# Autodesk Inventor assembly: deskShelf
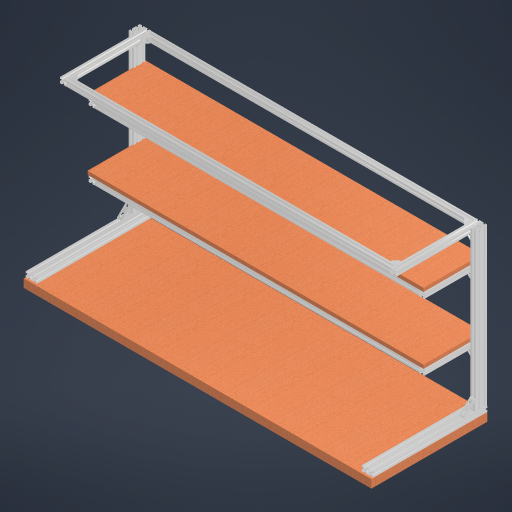
[picture p0: Inventor's stored thumbnail of the model, 512x512]
Saved by Autodesk Inventor 2023 (Build 270158000, 158)
## iProperties
Created: 2023-03-26
Part Number: deskShelf
Document SubType Name: Assembly
Designer: austi
Author: austi
## Documents named in this file (11)
- E:\OneDrive\work\deepSpaceEngineering\deskShelf.iam
- E:\OneDrive\work\deepSpaceEngineering\Part1.ipt
- E:\OneDrive\work\deepSpaceEngineering\shelf.ipt
- E:\OneDrive\work\deepSpaceEngineering\30-3030-1708-CL.ipt
- E:\OneDrive\work\deepSpaceEngineering\30-3060-825-CL.ipt
- E:\OneDrive\work\deepSpaceEngineering\30-3060-600-CL.ipt
- E:\OneDrive\work\deepSpaceEngineering\30-3030-300-CL.ipt
- E:\OneDrive\work\deepSpaceEngineering\30-3030-450-CL.ipt
- E:\OneDrive\work\deepSpaceEngineering\30-4336_Aluminum.ipt
- E:\OneDrive\work\deepSpaceEngineering\30-4134_Aluminum.ipt
- E:\OneDrive\work\deepSpaceEngineering\14073.ipt
## Components (39 placed, 10 different names)
1. Part1:1 — Mate:1, Flush:2, Flush:3, Mate:2, Mate:6, Mate:8, Flush:32
2. shelf:1 — Mate:63, Flush:51, Flush:52
3. shelf:2 — Mate:62, Flush:49, Flush:50
4. 30-3030-1708-CL:1 — Mate:11, Flush:12, Flush:13, Mate:49, Flush:42, Mate:56, Flush:46, Flush:49
5. 30-3030-1708-CL:2 — Flush:10, Mate:9, Flush:11, Mate:10, Flush:37, Mate:39, Mate:51, Mate:62
6. 30-3030-1708-CL:4 — Mate:17, Flush:18, Flush:19, Mate:47, Flush:41, Mate:58, Flush:47, Mate:63, Flush:52
7. 30-3030-1708-CL:6 — Mate:16, Flush:16, Flush:17, Mate:41, Mate:53
8. 30-3060-825-CL:1 — Mate:3, Flush:4, Flush:5, Mate:5, Flush:8, Mate:12, Flush:14, Mate:18, Flush:20, Flush:21, Mate:23, Flush:28, Mate:26, Mate:28, Flush:31, Mate:30
9. 30-3060-825-CL:2 — Mate:4, Flush:6, Flush:7, Flush:9, Mate:7, Mate:14, Flush:15, Mate:19, Flush:22, Flush:23, Mate:25, Flush:29, Mate:32, Flush:34, Mate:34, Flush:35, Mate:36, Flush:36
10. 30-3060-600-CL:1 — Mate:1, Flush:2, Mate:3, Flush:4, Flush:5, Mate:22, Flush:32
11. 30-3060-600-CL:2 — Flush:3, Mate:2, Mate:4, Flush:6, Flush:7, Mate:24
12. 30-3030-300-CL:1 — Mate:5, Flush:8, Mate:6, Mate:10, Mate:11, Flush:12, Flush:13, Mate:13, Mate:27, Flush:30, Mate:38, Mate:48, Flush:50
13. 30-3030-300-CL:2 — Mate:14, Flush:15, Mate:15, Mate:16, Flush:16, Flush:17, Mate:17, Flush:18, Flush:19, Mate:35, Mate:52, Flush:44, Mate:59
14. 30-3030-300-CL:3 — Mate:12, Flush:14, Mate:13, Mate:29, Mate:40, Flush:38, Mate:46, Flush:51
15. 30-3030-300-CL:4 — Flush:9, Mate:7, Mate:8, Flush:10, Mate:9, Flush:11, Mate:15, Mate:33, Mate:50, Flush:43, Mate:57
16. 30-3030-450-CL:1 — Mate:18, Flush:20, Flush:21, Mate:20, Flush:24, Flush:25, Mate:21, Flush:26, Flush:27, Mate:31, Flush:33, Mate:42, Flush:39, Mate:44
17. 30-3030-450-CL:2 — Mate:19, Flush:22, Flush:23, Mate:37, Mate:54, Flush:45, Mate:61
18. 30-3030-1708-CL:7 — Mate:21, Flush:26, Flush:27, Mate:43, Mate:55
19. 30-3030-1708-CL:8 — Mate:20, Flush:24, Flush:25, Mate:45, Flush:40, Mate:60, Flush:48
20. 30-4336_Aluminum:1 — Mate:22, Mate:23, Flush:28
21. 30-4336_Aluminum:2 — Mate:24, Mate:25, Flush:29
22. 30-4134_Aluminum:1 — Mate:32, Mate:33, Flush:34
23. 30-4134_Aluminum:2 — Mate:34, Mate:35, Flush:35
24. 30-4134_Aluminum:3 — Mate:36, Mate:37, Flush:36
25. 30-4134_Aluminum:4 — Mate:30, Mate:31, Flush:33
26. 30-4134_Aluminum:5 — Mate:28, Flush:31, Mate:29
27. 30-4134_Aluminum:6 — Mate:26, Mate:27, Flush:30
28. 14073:1 — Mate:38, Flush:37, Mate:39
29. 14073:2 — Mate:40, Flush:38, Mate:41
30. 14073:3 — Mate:42, Flush:39, Mate:43
31. 14073:4 — Mate:50, Mate:51, Flush:43
32. 14073:5 — Mate:52, Mate:53, Flush:44
33. 14073:6 — Mate:54, Mate:55, Flush:45
34. 14073:7 — Mate:56, Mate:57, Flush:46
35. 14073:8 — Mate:58, Mate:59, Flush:47
36. 14073:9 — Mate:60, Mate:61, Flush:48
37. 14073:10 — Mate:44, Mate:45, Flush:40
38. 14073:11 — Mate:48, Mate:49, Flush:42
39. 14073:12 — Mate:46, Mate:47, Flush:41
## Relationships (114: Mate 63, Flush 51)
- Mate:1: Part1:1 ↔ 30-3060-600-CL:1
- Flush:2: Part1:1 ↔ 30-3060-600-CL:1
- Flush:3: Part1:1 ↔ 30-3060-600-CL:2
- Mate:2: Part1:1 ↔ 30-3060-600-CL:2
- Mate:3: 30-3060-825-CL:1 ↔ 30-3060-600-CL:1
- Flush:4: 30-3060-825-CL:1 ↔ 30-3060-600-CL:1
- Flush:5: 30-3060-825-CL:1 ↔ 30-3060-600-CL:1
- Mate:4: 30-3060-825-CL:2 ↔ 30-3060-600-CL:2
- Flush:6: 30-3060-825-CL:2 ↔ 30-3060-600-CL:2
- Flush:7: 30-3060-825-CL:2 ↔ 30-3060-600-CL:2
- Mate:5: 30-3060-825-CL:1 ↔ 30-3030-300-CL:1
- Flush:8: 30-3060-825-CL:1 ↔ 30-3030-300-CL:1
- Mate:6 (300 mm): Part1:1 ↔ 30-3030-300-CL:1
- Flush:9: 30-3060-825-CL:2 ↔ 30-3030-300-CL:4
- Mate:7: 30-3060-825-CL:2 ↔ 30-3030-300-CL:4
- Mate:8 (300 mm): Part1:1 ↔ 30-3030-300-CL:4
- Flush:10: 30-3030-1708-CL:2 ↔ 30-3030-300-CL:4
- Mate:9: 30-3030-1708-CL:2 ↔ 30-3030-300-CL:4
- Flush:11: 30-3030-1708-CL:2 ↔ 30-3030-300-CL:4
- Mate:10: 30-3030-1708-CL:2 ↔ 30-3030-300-CL:1
- Mate:11: 30-3030-1708-CL:1 ↔ 30-3030-300-CL:1
- Flush:12: 30-3030-1708-CL:1 ↔ 30-3030-300-CL:1
- Flush:13: 30-3030-1708-CL:1 ↔ 30-3030-300-CL:1
- Mate:12: 30-3060-825-CL:1 ↔ 30-3030-300-CL:3
- Flush:14: 30-3060-825-CL:1 ↔ 30-3030-300-CL:3
- Mate:13 (320 mm): 30-3030-300-CL:1 ↔ 30-3030-300-CL:3
- Mate:14: 30-3060-825-CL:2 ↔ 30-3030-300-CL:2
- Flush:15: 30-3060-825-CL:2 ↔ 30-3030-300-CL:2
- Mate:15 (320 mm): 30-3030-300-CL:2 ↔ 30-3030-300-CL:4
- Mate:16: 30-3030-1708-CL:6 ↔ 30-3030-300-CL:2
- Flush:16: 30-3030-1708-CL:6 ↔ 30-3030-300-CL:2
- Flush:17: 30-3030-1708-CL:6 ↔ 30-3030-300-CL:2
- Mate:17: 30-3030-1708-CL:4 ↔ 30-3030-300-CL:2
- Flush:18: 30-3030-1708-CL:4 ↔ 30-3030-300-CL:2
- Flush:19: 30-3030-1708-CL:4 ↔ 30-3030-300-CL:2
- Mate:18: 30-3060-825-CL:1 ↔ 30-3030-450-CL:1
- Flush:20: 30-3060-825-CL:1 ↔ 30-3030-450-CL:1
- Flush:21: 30-3060-825-CL:1 ↔ 30-3030-450-CL:1
- Mate:19: 30-3060-825-CL:2 ↔ 30-3030-450-CL:2
- Flush:22: 30-3060-825-CL:2 ↔ 30-3030-450-CL:2
- Flush:23: 30-3060-825-CL:2 ↔ 30-3030-450-CL:2
- Mate:20: 30-3030-450-CL:1 ↔ 30-3030-1708-CL:8
- Flush:24: 30-3030-450-CL:1 ↔ 30-3030-1708-CL:8
- Flush:25: 30-3030-450-CL:1 ↔ 30-3030-1708-CL:8
- Mate:21: 30-3030-450-CL:1 ↔ 30-3030-1708-CL:7
- Flush:26: 30-3030-450-CL:1 ↔ 30-3030-1708-CL:7
- Flush:27: 30-3030-450-CL:1 ↔ 30-3030-1708-CL:7
- Mate:22: 30-3060-600-CL:1 ↔ 30-4336_Aluminum:1
- Mate:23: 30-3060-825-CL:1 ↔ 30-4336_Aluminum:1
- Flush:28: 30-3060-825-CL:1 ↔ 30-4336_Aluminum:1
- Mate:24: 30-3060-600-CL:2 ↔ 30-4336_Aluminum:2
- Mate:25: 30-3060-825-CL:2 ↔ 30-4336_Aluminum:2
- Flush:29: 30-3060-825-CL:2 ↔ 30-4336_Aluminum:2
- Mate:26: 30-3060-825-CL:1 ↔ 30-4134_Aluminum:6
- Mate:27: 30-3030-300-CL:1 ↔ 30-4134_Aluminum:6
- Flush:30: 30-3030-300-CL:1 ↔ 30-4134_Aluminum:6
- Mate:28: 30-3060-825-CL:1 ↔ 30-4134_Aluminum:5
- Flush:31: 30-3060-825-CL:1 ↔ 30-4134_Aluminum:5
- Flush:32: Part1:1 ↔ 30-3060-600-CL:1
- Mate:29: 30-3030-300-CL:3 ↔ 30-4134_Aluminum:5
- Mate:30: 30-3060-825-CL:1 ↔ 30-4134_Aluminum:4
- Mate:31: 30-3030-450-CL:1 ↔ 30-4134_Aluminum:4
- Flush:33: 30-3030-450-CL:1 ↔ 30-4134_Aluminum:4
- Mate:32: 30-3060-825-CL:2 ↔ 30-4134_Aluminum:1
- Mate:33: 30-3030-300-CL:4 ↔ 30-4134_Aluminum:1
- Flush:34: 30-3060-825-CL:2 ↔ 30-4134_Aluminum:1
- Mate:34: 30-3060-825-CL:2 ↔ 30-4134_Aluminum:2
- Mate:35: 30-3030-300-CL:2 ↔ 30-4134_Aluminum:2
- Flush:35: 30-3060-825-CL:2 ↔ 30-4134_Aluminum:2
- Mate:36: 30-3060-825-CL:2 ↔ 30-4134_Aluminum:3
- Mate:37: 30-3030-450-CL:2 ↔ 30-4134_Aluminum:3
- Flush:36: 30-3060-825-CL:2 ↔ 30-4134_Aluminum:3
- Mate:38: 30-3030-300-CL:1 ↔ 14073:1
- Flush:37: 30-3030-1708-CL:2 ↔ 14073:1
- Mate:39: 30-3030-1708-CL:2 ↔ 14073:1
- Mate:40: 30-3030-300-CL:3 ↔ 14073:2
- Flush:38: 30-3030-300-CL:3 ↔ 14073:2
- Mate:41: 30-3030-1708-CL:6 ↔ 14073:2
- Mate:42: 30-3030-450-CL:1 ↔ 14073:3
- Flush:39: 30-3030-450-CL:1 ↔ 14073:3
- Mate:43: 30-3030-1708-CL:7 ↔ 14073:3
- Mate:44: 30-3030-450-CL:1 ↔ 14073:10
- Mate:45: 30-3030-1708-CL:8 ↔ 14073:10
- Flush:40: 30-3030-1708-CL:8 ↔ 14073:10
- Mate:46: 30-3030-300-CL:3 ↔ 14073:12
- Mate:47: 30-3030-1708-CL:4 ↔ 14073:12
- Flush:41: 30-3030-1708-CL:4 ↔ 14073:12
- Mate:48: 30-3030-300-CL:1 ↔ 14073:11
- Mate:49: 30-3030-1708-CL:1 ↔ 14073:11
- Flush:42: 30-3030-1708-CL:1 ↔ 14073:11
- Mate:50: 30-3030-300-CL:4 ↔ 14073:4
- Mate:51: 30-3030-1708-CL:2 ↔ 14073:4
- Flush:43: 30-3030-300-CL:4 ↔ 14073:4
- Mate:52: 30-3030-300-CL:2 ↔ 14073:5
- Mate:53: 30-3030-1708-CL:6 ↔ 14073:5
- Flush:44: 30-3030-300-CL:2 ↔ 14073:5
- Mate:54: 30-3030-450-CL:2 ↔ 14073:6
- Mate:55: 30-3030-1708-CL:7 ↔ 14073:6
- Flush:45: 30-3030-450-CL:2 ↔ 14073:6
- Mate:56: 30-3030-1708-CL:1 ↔ 14073:7
- Mate:57: 30-3030-300-CL:4 ↔ 14073:7
- Flush:46: 30-3030-1708-CL:1 ↔ 14073:7
- Mate:58: 30-3030-1708-CL:4 ↔ 14073:8
- Mate:59: 30-3030-300-CL:2 ↔ 14073:8
- Flush:47: 30-3030-1708-CL:4 ↔ 14073:8
- Mate:60: 30-3030-1708-CL:8 ↔ 14073:9
- Mate:61: 30-3030-450-CL:2 ↔ 14073:9
- Flush:48: 30-3030-1708-CL:8 ↔ 14073:9
- Mate:62: shelf:2 ↔ 30-3030-1708-CL:2
- Flush:49: shelf:2 ↔ 30-3030-1708-CL:1
- Flush:50: shelf:2 ↔ 30-3030-300-CL:1
- Mate:63: shelf:1 ↔ 30-3030-1708-CL:4
- Flush:51: shelf:1 ↔ 30-3030-300-CL:3
- Flush:52: shelf:1 ↔ 30-3030-1708-CL:4
